# Autodesk Inventor assembly: G
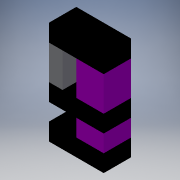
[picture p0: Inventor's stored thumbnail of the model, 180x180]
Saved by Autodesk Inventor 2016 (Build 200138000, 138)
## iProperties
Created: 2016-07-21
Part Number: G
Document SubType Name: Assembly
Designer: cfkguest
Author: cfkguest
## Documents named in this file (4)
- E:\Austin Abraham\College For Kids (CFK)\AIT Building\3) Computer Aided Design & Drafting (CAD)\Autodesk\Autodesk Inventor\Legos\G.iam
- E:\Austin Abraham\College For Kids (CFK)\AIT Building\3) Computer Aided Design & Drafting (CAD)\Autodesk\Autodesk Inventor\Legos\4 x2.ipt
- E:\Austin Abraham\College For Kids (CFK)\AIT Building\3) Computer Aided Design & Drafting (CAD)\Autodesk\Autodesk Inventor\Legos\2 x2.ipt
- E:\Austin Abraham\College For Kids (CFK)\AIT Building\3) Computer Aided Design & Drafting (CAD)\Autodesk\Autodesk Inventor\Legos\2 x1.ipt
## Components (8 placed, 3 different names)
1. 4 x2:1 — Mate:1, Flush:1, Flush:2
2. 2 x2:1 — Mate:1, Flush:1, Flush:2, Mate:2, Flush:3, Flush:4
3. 4 x2:2 — Mate:2, Flush:3, Flush:4, Mate:4, Flush:7, Flush:8, Mate:5, Flush:9, Flush:10
4. 2 x1:1 — Mate:3, Flush:5, Flush:6, Mate:4, Flush:7, Flush:8
5. 2 x1:2 — Mate:3, Flush:5, Flush:6
6. 2 x2:2 — Mate:5, Flush:9, Flush:10, Flush:11, Flush:12, Mate:6
7. 2 x2:3 — Flush:11, Flush:12, Mate:6, Flush:13, Flush:14, Mate:7
8. 4 x2:3 — Flush:13, Flush:14, Mate:7
## Relationships (21: Flush 14, Mate 7)
- Mate:1: 4 x2:1 ↔ 2 x2:1
- Flush:1: 4 x2:1 ↔ 2 x2:1
- Flush:2: 4 x2:1 ↔ 2 x2:1
- Mate:2: 2 x2:1 ↔ 4 x2:2
- Flush:3: 2 x2:1 ↔ 4 x2:2
- Flush:4: 2 x2:1 ↔ 4 x2:2
- Mate:3: 2 x1:1 ↔ 2 x1:2
- Flush:5: 2 x1:1 ↔ 2 x1:2
- Flush:6: 2 x1:1 ↔ 2 x1:2
- Mate:4: 4 x2:2 ↔ 2 x1:1
- Flush:7: 4 x2:2 ↔ 2 x1:1
- Flush:8: 4 x2:2 ↔ 2 x1:1
- Mate:5: 4 x2:2 ↔ 2 x2:2
- Flush:9: 4 x2:2 ↔ 2 x2:2
- Flush:10: 4 x2:2 ↔ 2 x2:2
- Flush:11: 2 x2:2 ↔ 2 x2:3
- Flush:12: 2 x2:2 ↔ 2 x2:3
- Mate:6: 2 x2:2 ↔ 2 x2:3
- Flush:13: 2 x2:3 ↔ 4 x2:3
- Flush:14: 2 x2:3 ↔ 4 x2:3
- Mate:7: 2 x2:3 ↔ 4 x2:3
